# Autodesk Inventor assembly: Base
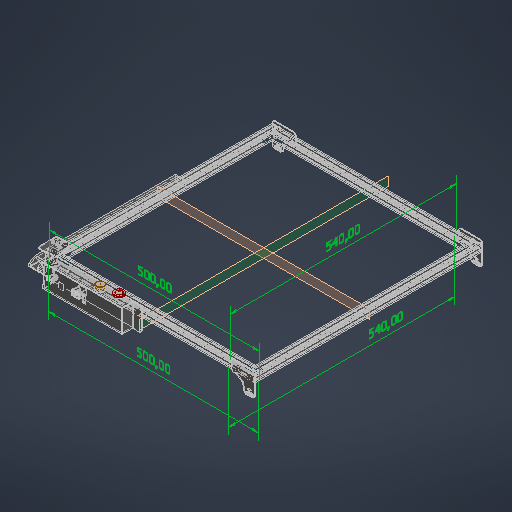
[picture p0: Inventor's stored thumbnail of the model, 512x512]
Saved by Autodesk Inventor 2025 (Build 290162000, 162)
## iProperties
Created: 2024-11-17
Part Number: Base
Document SubType Name: Assembly
Designer: Admin
Author: Admin
Revision Number: ANY
## Documents named in this file (21)
- V:\INVENTOR\laser\ortur\ortur_laser_master_s2_information\inventor\Ortur Laser Master 2 Pro S2 LF\Base.iam
- V:\INVENTOR\laser\ortur\ortur_laser_master_s2_information\inventor\Ortur Laser Master 2 Pro S2 LF\plain washer 6902 type abc_din_DIN 6902-A5.5.ipt
- V:\INVENTOR\laser\ortur\ortur_laser_master_s2_information\inventor\Ortur Laser Master 2 Pro S2 LF\Vis cruci_DIN EN ISO 7045 - M5 x 10 - Z - 10N.ipt
- V:\INVENTOR\laser\ortur\ortur_laser_master_s2_information\inventor\Ortur Laser Master 2 Pro S2 LF\Vis cruci_DIN EN ISO 7045 - M5 x 30 - Z - 30N.ipt
- V:\INVENTOR\laser\ortur\ortur_laser_master_s2_information\inventor\Ortur Laser Master 2 Pro S2 LF\Vis cruci_DIN EN ISO 7045 - M2 x 10 - Z - 10N.ipt
- V:\INVENTOR\laser\ortur\ortur_laser_master_s2_information\inventor\Ortur Laser Master 2 Pro S2 LF\Profilé 540mm.ipt
- V:\INVENTOR\laser\ortur\ortur_laser_master_s2_information\inventor\Ortur Laser Master 2 Pro S2 LF\Profilé 460mm.ipt
- V:\INVENTOR\laser\ortur\ortur_laser_master_s2_information\inventor\Ortur Laser Master 2 Pro S2 LF\Pied.ipt
- V:\INVENTOR\laser\ortur\ortur_laser_master_s2_information\inventor\Ortur Laser Master 2 Pro S2 LF\Support capteur Y.ipt
- V:\INVENTOR\laser\ortur\ortur_laser_master_s2_information\inventor\Ortur Laser Master 2 Pro S2 LF\Microswitch Omron SS-5GL-F.ipt
- V:\INVENTOR\laser\ortur\ortur_laser_master_s2_information\inventor\Ortur Laser Master 2 Pro S2 LF\Panneau de controle.ipt
- V:\INVENTOR\laser\ortur\ortur_laser_master_s2_information\inventor\Ortur Laser Master 2 Pro S2 LF\connecteur 2x9.ipt
- V:\INVENTOR\laser\ortur\ortur_laser_master_s2_information\inventor\Ortur Laser Master 2 Pro S2 LF\connecteur 2x5.ipt
- V:\INVENTOR\laser\ortur\ortur_laser_master_s2_information\inventor\Ortur Laser Master 2 Pro S2 LF\PJ-102BH.ipt
- V:\INVENTOR\laser\ortur\ortur_laser_master_s2_information\inventor\Ortur Laser Master 2 Pro S2 LF\USB 2.0 Type B Connector Right Angle (Würth 61400416121).ipt
- V:\INVENTOR\laser\ortur\ortur_laser_master_s2_information\inventor\Ortur Laser Master 2 Pro S2 LF\RJ11_Female_Connector.ipt
- V:\INVENTOR\laser\ortur\ortur_laser_master_s2_information\inventor\Ortur Laser Master 2 Pro S2 LF\connecteur 2x3.ipt
- V:\INVENTOR\laser\ortur\ortur_laser_master_s2_information\inventor\Ortur Laser Master 2 Pro S2 LF\Mousse pieds.ipt
- V:\INVENTOR\laser\ortur\ortur_laser_master_s2_information\inventor\Ortur Laser Master 2 Pro S2 LF\2020_int_L_joint___ _________.ipt
- V:\INVENTOR\laser\ortur\ortur_laser_master_s2_information\inventor\Ortur Laser Master 2 Pro S2 LF\Support chaine.ipt
- V:\INVENTOR\laser\ortur\ortur_laser_master_s2_information\inventor\Ortur Laser Master 2 Pro S2 LF\Chaine porte cable 1_350.ipt
## Components (42 placed, 42 different names)
1. plain washer 6902 type abc_din_DIN 6902-A5.5_199
2. Vis cruci_DIN EN ISO 7045 - M5 x 10 - Z - 10N_200
3. Vis cruci_DIN EN ISO 7045 - M5 x 30 - Z - 30N_201
4. plain washer 6902 type abc_din_DIN 6902-A5.5_202
5. plain washer 6902 type abc_din_DIN 6902-A5.5_203
6. Vis cruci_DIN EN ISO 7045 - M5 x 30 - Z - 30N_204
7. Vis cruci_DIN EN ISO 7045 - M5 x 10 - Z - 10N_205
8. Vis cruci_DIN EN ISO 7045 - M5 x 30 - Z - 30N_206
9. Vis cruci_DIN EN ISO 7045 - M5 x 10 - Z - 10N_207
10. Vis cruci_DIN EN ISO 7045 - M2 x 10 - Z - 10N_208
11. Vis cruci_DIN EN ISO 7045 - M2 x 10 - Z - 10N_209
12. Vis cruci_DIN EN ISO 7045 - M5 x 10 - Z - 10N_210
13. Vis cruci_DIN EN ISO 7045 - M5 x 10 - Z - 10N_211
14. Vis cruci_DIN EN ISO 7045 - M5 x 10 - Z - 10N_214
15. Vis cruci_DIN EN ISO 7045 - M5 x 10 - Z - 10N_215
16. Vis cruci_DIN EN ISO 7045 - M5 x 30 - Z - 30N_216
17. Profilé 540mm_217 — Symmetry:2
18. Profilé 460mm_218 — Symmetry:1
19. Profilé 540mm_219 — Symmetry:2
20. Profilé 460mm_220 — Symmetry:1
21. Pied_221
22. Pied_222
23. Pied_223
24. Support capteur Y_224
25. Microswitch Omron SS-5GL-F_225
26. Panneau de controle_226
27. connecteur 2x9_227
28. connecteur 2x5_228
29. PJ-102BH_229
30. USB 2.0 Type B Connector Right Angle (Würth 61400416121)_230
31. RJ11_Female_Connector_231
32. connecteur 2x3_232
33. Mousse pieds_235
34. Mousse pieds_236
35. Mousse pieds_237
36. Mousse pieds_238
37. 2020_int_L_joint___ __________239
38. 2020_int_L_joint___ __________240
39. 2020_int_L_joint___ __________241
40. 2020_int_L_joint___ __________242
41. Support chaine_243
42. Chaine porte cable 1_350_244
## Relationships (2: Symmetry 2)
- Symmetry:1: Profilé 460mm_218 ↔ Profilé 460mm_220
- Symmetry:2: Profilé 540mm_217 ↔ Profilé 540mm_219
